# Autodesk Inventor assembly: MechanumChassis
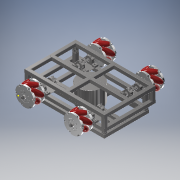
[picture p0: Inventor's stored thumbnail of the model, 180x180]
Saved by Autodesk Inventor 2018 (Build 220112000, 112)
## iProperties
Created: 2017-10-18
Part Number: MechanumChassis
Document SubType Name: Weldment
Designer: Bryce Richards
Mass: 42172.1 g
Surface Area: 44852.8 cm^2
Volume: 5448.29 cm^3
Density: 7.74044 g/cm^3
Weld Material: Steel, Mild, Welded
Author: Bryce Richards
## Documents named in this file (18)
- C:\Users\P136265\Documents\mecanum-cad\MechanumChassis.iam
- C:\Users\P136265\Documents\mecanum-cad\MecanumFrame2.iam
- C:\Users\P136265\Documents\mecanum-cad\PillowAssembly.iam
- C:\Users\P136265\Documents\Inventor\Content Center Files\R2018\en-US\AS 1110\AS 1110 - M8 x 60.ipt
- C:\Users\P136265\Documents\Inventor\Content Center Files\R2018\en-US\AS 1112 (2)\AS 1112 - M8  Type 5.ipt
- C:\Users\P136265\Documents\mecanum-cad\PillowPlate.ipt
- C:\Users\P136265\Documents\mecanum-cad\LiftPlate.iam
- C:\Users\P136265\Documents\mecanum-cad\AlignmentTube.ipt
- C:\Users\P136265\Documents\mecanum-cad\LoadTestBlock.ipt
- C:\Users\P136265\Documents\mecanum-cad\WheelShaft.ipt
- C:\Users\P136265\Documents\mecanum-cad\Mecanum_Assembly.iam
- C:\Users\P136265\Documents\Inventor\Content Center Files\R2018\en-US\ISO 4032(2)\ISO 4032 - M20 - ISO.ipt
- C:\Users\P136265\Documents\mecanum-cad\MechanumChassis\AIP\FEA\cayefugao.fins
- C:\Users\P136265\Documents\mecanum-cad\MechanumChassis\AIP\FEA\cayefugao.fsat
- C:\Users\P136265\Documents\mecanum-cad\MechanumChassis\AIP\FEA\cayefugao.ftes
- C:\Users\P136265\Documents\mecanum-cad\MechanumChassis\AIP\FEA\cayefugao.fwiz
- C:\Users\P136265\Documents\mecanum-cad\MechanumChassis\AIP\FEA\cayefuglc.fmsh
- C:\Users\P136265\Documents\mecanum-cad\MechanumChassis\AIP\FEA\cayefugld.fres
## Components (67 placed, 11 different names)
1. MecanumFrame2:1 [sub-assembly] — Flush:2, Flush:6, Flush:7, Mate:56, Mate:69, Mate:70, Mate:71, Mate:90, Angle:5, Angle:6, Angle:7, Flush:10, Insert:17, Insert:18, Insert:19, Insert:20, Insert:21, Insert:22, Insert:23, Insert:24, Insert:25, Insert:26, Insert:27, Insert:28, Insert:29, Insert:30, Insert:31, Insert:32, Angle:8, Mate:209, Mate:210, Flush:11, Angle:9, Angle:10, Angle:11, Mate:211, Mate:212, Flush:12, Mate:213, Mate:214, Flush:13, Mate:215, Mate:216, Flush:14, Angle:12, Mate:221, Mate:222, Mate:223, Angle:13, Angle:14, Angle:15, Angle:16, Angle:17, Angle:18, Angle:19, Angle:20, Mate:225, Mate:226, Mate:227, Mate:228, Mate:234, Mate:235, Mate:236, Mate:237
2. PillowAssembly:1 [sub-assembly] — Mate:16, Mate:59, Mate:186, Mate:190, Mate:233, Flush:17, Mate:234
3. PillowAssembly:2 [sub-assembly] — Mate:13, Mate:62, Mate:178, Mate:180, Mate:231, Mate:232, Mate:235
4. PillowAssembly:3 [sub-assembly] — Mate:15, Mate:63, Mate:64, Mate:202, Mate:206, Mate:230, Flush:16, Mate:236
5. PillowAssembly:4 [sub-assembly] — Mate:51, Mate:52, Mate:53, Mate:194, Mate:196, Mate:229, Flush:15, Mate:237
6. PillowAssembly:5 [sub-assembly] — Mate:13, Flush:2, Mate:60, Mate:61, Mate:182, Mate:184, Mate:253
7. PillowAssembly:6 [sub-assembly] — Mate:15, Mate:65, Flush:10, Mate:204, Mate:208, Mate:251
8. PillowAssembly:7 [sub-assembly] — Flush:6, Mate:16, Mate:57, Mate:58, Mate:188, Mate:192, Mate:257
9. PillowAssembly:8 [sub-assembly] — Flush:7, Mate:51, Mate:54, Mate:198, Mate:200, Mate:255
10. PillowPlate:1 — Mate:52, Mate:53, Mate:54, Mate:56
11. PillowPlate:2 — Mate:57, Mate:58, Mate:59, Mate:71
12. PillowPlate:3 — Mate:60, Mate:61, Mate:62, Mate:70
13. PillowPlate:4 — Mate:63, Mate:64, Mate:65, Mate:69
14. LiftPlate:1 [sub-assembly] — Angle:13, Angle:14, Angle:15, Angle:16, Angle:17, Angle:18, Angle:19, Angle:20, Mate:225, Mate:226, Mate:227, Mate:228
15. AS 1110 - Metric M8 x 60:17 — Insert:17, Mate:179
16. AS 1110 - Metric M8 x 60:18 — Insert:18, Mate:177
17. AS 1110 - Metric M8 x 60:19 — Insert:19, Mate:183
18. AS 1110 - Metric M8 x 60:20 — Insert:20, Mate:181
19. AS 1110 - Metric M8 x 60:21 — Insert:21, Mate:187
20. AS 1110 - Metric M8 x 60:22 — Insert:22, Mate:191
21. AS 1110 - Metric M8 x 60:23 — Insert:23, Mate:189
22. AS 1110 - Metric M8 x 60:24 — Insert:24, Mate:185
23. AS 1110 - Metric M8 x 60:25 — Insert:25, Mate:199
24. AS 1110 - Metric M8 x 60:26 — Insert:26, Mate:197
25. AS 1110 - Metric M8 x 60:27 — Insert:27, Mate:195
26. AS 1110 - Metric M8 x 60:28 — Insert:28, Mate:193
27. AS 1110 - Metric M8 x 60:29 — Insert:29, Mate:201
28. AS 1110 - Metric M8 x 60:30 — Insert:30, Mate:203
29. AS 1110 - Metric M8 x 60:31 — Insert:31, Mate:207
30. AS 1110 - Metric M8 x 60:32 — Insert:32, Mate:205
31. AS 1112 (2) - Metric M8  Type 5:17 — Mate:177, Mate:178
32. AS 1112 (2) - Metric M8  Type 5:18 — Mate:179, Mate:180
33. AS 1112 (2) - Metric M8  Type 5:19 — Mate:181, Mate:182
34. AS 1112 (2) - Metric M8  Type 5:20 — Mate:183, Mate:184
35. AS 1112 (2) - Metric M8  Type 5:21 — Mate:185, Mate:186
36. AS 1112 (2) - Metric M8  Type 5:22 — Mate:187, Mate:188
37. AS 1112 (2) - Metric M8  Type 5:23 — Mate:189, Mate:190
38. AS 1112 (2) - Metric M8  Type 5:24 — Mate:191, Mate:192
39. AS 1112 (2) - Metric M8  Type 5:25 — Mate:193, Mate:194
40. AS 1112 (2) - Metric M8  Type 5:26 — Mate:195, Mate:196
41. AS 1112 (2) - Metric M8  Type 5:27 — Mate:197, Mate:198
42. AS 1112 (2) - Metric M8  Type 5:28 — Mate:199, Mate:200
43. AS 1112 (2) - Metric M8  Type 5:29 — Mate:201, Mate:202
44. AS 1112 (2) - Metric M8  Type 5:30 — Mate:203, Mate:204
45. AS 1112 (2) - Metric M8  Type 5:31 — Mate:205, Mate:206
46. AS 1112 (2) - Metric M8  Type 5:32 — Mate:207, Mate:208
47. LoadTestBlock:1 — Angle:12, Mate:221, Mate:222, Mate:223
48. AlignmentTube:1 — Angle:10, Mate:213, Mate:214, Flush:13
49. AlignmentTube:2 — Angle:8, Mate:209, Mate:210, Flush:11
50. AlignmentTube:3 — Angle:11, Mate:215, Mate:216, Flush:14
51. AlignmentTube:4 — Angle:9, Mate:211, Mate:212, Flush:12
52. WheelShaft:1 — Mate:233, Flush:17, Angle:23, Angle:26, Mate:240, Flush:20, Mate:244, Mate:256
53. WheelShaft:2 — Mate:231, Mate:232, Angle:22, Angle:27, Mate:241, Flush:21, Mate:242, Mate:252
54. WheelShaft:3 — Mate:230, Flush:16, Angle:21, Angle:22, Angle:23, Angle:25, Mate:239, Flush:19, Mate:246, Mate:250
55. WheelShaft:4 — Mate:229, Flush:15, Angle:21, Angle:24, Mate:238, Flush:18, Mate:248, Mate:254
56. Mecanum_Assembly:1 [sub-assembly] — Angle:27, Mate:241, Flush:21, Mate:243
57. Mecanum_Assembly:2 [sub-assembly] — Angle:26, Mate:240, Flush:20, Mate:245
58. Mecanum_Assembly:3 [sub-assembly] — Angle:25, Mate:239, Flush:19, Mate:247
59. Mecanum_Assembly:4 [sub-assembly] — Angle:24, Mate:238, Flush:18, Mate:249
60. ISO 4032 M20:1 — Mate:242, Mate:243
61. ISO 4032 M20:2 — Mate:244, Mate:245
62. ISO 4032 M20:3 — Mate:246, Mate:247
63. ISO 4032 M20:4 — Mate:248, Mate:249
64. ISO 4032 M20:5 — Mate:250, Mate:251
65. ISO 4032 M20:6 — Mate:252, Mate:253
66. ISO 4032 M20:7 — Mate:254, Mate:255
67. ISO 4032 M20:8 — Mate:256, Mate:257
## Relationships (151: Mate 97, Angle 23, Insert 16, Flush 15)
- Mate:13: PillowAssembly:2 ↔ PillowAssembly:5
- Flush:2: MecanumFrame2:1 ↔ PillowAssembly:5
- Mate:15: PillowAssembly:3 ↔ PillowAssembly:6
- Flush:6: MecanumFrame2:1 ↔ PillowAssembly:7
- Mate:16: PillowAssembly:1 ↔ PillowAssembly:7
- Flush:7: MecanumFrame2:1 ↔ PillowAssembly:8
- Mate:51: PillowAssembly:4 ↔ PillowAssembly:8
- Mate:52: PillowAssembly:4 ↔ PillowPlate:1
- Mate:53: PillowAssembly:4 ↔ PillowPlate:1
- Mate:54: PillowAssembly:8 ↔ PillowPlate:1
- Mate:56: MecanumFrame2:1 ↔ PillowPlate:1
- Mate:57: PillowAssembly:7 ↔ PillowPlate:2
- Mate:58: PillowAssembly:7 ↔ PillowPlate:2
- Mate:59: PillowAssembly:1 ↔ PillowPlate:2
- Mate:60: PillowAssembly:5 ↔ PillowPlate:3
- Mate:61: PillowAssembly:5 ↔ PillowPlate:3
- Mate:62: PillowAssembly:2 ↔ PillowPlate:3
- Mate:63: PillowAssembly:3 ↔ PillowPlate:4
- Mate:64: PillowAssembly:3 ↔ PillowPlate:4
- Mate:65: PillowAssembly:6 ↔ PillowPlate:4
- Mate:69: MecanumFrame2:1 ↔ PillowPlate:4
- Mate:70: MecanumFrame2:1 ↔ PillowPlate:3
- Mate:71: MecanumFrame2:1 ↔ PillowPlate:2
- Mate:90: MecanumFrame2:1
- Angle:5 (0 deg): MecanumFrame2:1
- Angle:6 (0 deg): MecanumFrame2:1
- Angle:7 (0 deg): MecanumFrame2:1
- Flush:10: MecanumFrame2:1 ↔ PillowAssembly:6
- Insert:17: MecanumFrame2:1 ↔ AS 1110 - Metric M8 x 60:17
- Insert:18: MecanumFrame2:1 ↔ AS 1110 - Metric M8 x 60:18
- Insert:19: MecanumFrame2:1 ↔ AS 1110 - Metric M8 x 60:19
- Insert:20: MecanumFrame2:1 ↔ AS 1110 - Metric M8 x 60:20
- Insert:21: MecanumFrame2:1 ↔ AS 1110 - Metric M8 x 60:21
- Insert:22: MecanumFrame2:1 ↔ AS 1110 - Metric M8 x 60:22
- Insert:23: MecanumFrame2:1 ↔ AS 1110 - Metric M8 x 60:23
- Insert:24: MecanumFrame2:1 ↔ AS 1110 - Metric M8 x 60:24
- Insert:25: MecanumFrame2:1 ↔ AS 1110 - Metric M8 x 60:25
- Insert:26: MecanumFrame2:1 ↔ AS 1110 - Metric M8 x 60:26
- Insert:27: MecanumFrame2:1 ↔ AS 1110 - Metric M8 x 60:27
- Insert:28: MecanumFrame2:1 ↔ AS 1110 - Metric M8 x 60:28
- Insert:29: MecanumFrame2:1 ↔ AS 1110 - Metric M8 x 60:29
- Insert:30: MecanumFrame2:1 ↔ AS 1110 - Metric M8 x 60:30
- Insert:31: MecanumFrame2:1 ↔ AS 1110 - Metric M8 x 60:31
- Insert:32: MecanumFrame2:1 ↔ AS 1110 - Metric M8 x 60:32
- Mate:177: AS 1110 - Metric M8 x 60:18 ↔ AS 1112 (2) - Metric M8  Type 5:17
- Mate:178: PillowAssembly:2 ↔ AS 1112 (2) - Metric M8  Type 5:17
- Mate:179: AS 1110 - Metric M8 x 60:17 ↔ AS 1112 (2) - Metric M8  Type 5:18
- Mate:180: PillowAssembly:2 ↔ AS 1112 (2) - Metric M8  Type 5:18
- Mate:181: AS 1110 - Metric M8 x 60:20 ↔ AS 1112 (2) - Metric M8  Type 5:19
- Mate:182: PillowAssembly:5 ↔ AS 1112 (2) - Metric M8  Type 5:19
- Mate:183: AS 1110 - Metric M8 x 60:19 ↔ AS 1112 (2) - Metric M8  Type 5:20
- Mate:184: PillowAssembly:5 ↔ AS 1112 (2) - Metric M8  Type 5:20
- Mate:185: AS 1110 - Metric M8 x 60:24 ↔ AS 1112 (2) - Metric M8  Type 5:21
- Mate:186: PillowAssembly:1 ↔ AS 1112 (2) - Metric M8  Type 5:21
- Mate:187: AS 1110 - Metric M8 x 60:21 ↔ AS 1112 (2) - Metric M8  Type 5:22
- Mate:188: PillowAssembly:7 ↔ AS 1112 (2) - Metric M8  Type 5:22
- Mate:189: AS 1110 - Metric M8 x 60:23 ↔ AS 1112 (2) - Metric M8  Type 5:23
- Mate:190: PillowAssembly:1 ↔ AS 1112 (2) - Metric M8  Type 5:23
- Mate:191: AS 1110 - Metric M8 x 60:22 ↔ AS 1112 (2) - Metric M8  Type 5:24
- Mate:192: PillowAssembly:7 ↔ AS 1112 (2) - Metric M8  Type 5:24
- Mate:193: AS 1110 - Metric M8 x 60:28 ↔ AS 1112 (2) - Metric M8  Type 5:25
- Mate:194: PillowAssembly:4 ↔ AS 1112 (2) - Metric M8  Type 5:25
- Mate:195: AS 1110 - Metric M8 x 60:27 ↔ AS 1112 (2) - Metric M8  Type 5:26
- Mate:196: PillowAssembly:4 ↔ AS 1112 (2) - Metric M8  Type 5:26
- Mate:197: AS 1110 - Metric M8 x 60:26 ↔ AS 1112 (2) - Metric M8  Type 5:27
- Mate:198: PillowAssembly:8 ↔ AS 1112 (2) - Metric M8  Type 5:27
- Mate:199: AS 1110 - Metric M8 x 60:25 ↔ AS 1112 (2) - Metric M8  Type 5:28
- Mate:200: PillowAssembly:8 ↔ AS 1112 (2) - Metric M8  Type 5:28
- Mate:201: AS 1110 - Metric M8 x 60:29 ↔ AS 1112 (2) - Metric M8  Type 5:29
- Mate:202: PillowAssembly:3 ↔ AS 1112 (2) - Metric M8  Type 5:29
- Mate:203: AS 1110 - Metric M8 x 60:30 ↔ AS 1112 (2) - Metric M8  Type 5:30
- Mate:204: PillowAssembly:6 ↔ AS 1112 (2) - Metric M8  Type 5:30
- Mate:205: AS 1110 - Metric M8 x 60:32 ↔ AS 1112 (2) - Metric M8  Type 5:31
- Mate:206: PillowAssembly:3 ↔ AS 1112 (2) - Metric M8  Type 5:31
- Mate:207: AS 1110 - Metric M8 x 60:31 ↔ AS 1112 (2) - Metric M8  Type 5:32
- Mate:208: PillowAssembly:6 ↔ AS 1112 (2) - Metric M8  Type 5:32
- Angle:8 (0 deg): MecanumFrame2:1 ↔ AlignmentTube:2
- Mate:209: MecanumFrame2:1 ↔ AlignmentTube:2
- Mate:210: MecanumFrame2:1 ↔ AlignmentTube:2
- Flush:11: MecanumFrame2:1 ↔ AlignmentTube:2
- Angle:9 (0 deg): MecanumFrame2:1 ↔ AlignmentTube:4
- Angle:10 (0 deg): MecanumFrame2:1 ↔ AlignmentTube:1
- Angle:11 (0 deg): MecanumFrame2:1 ↔ AlignmentTube:3
- Mate:211: MecanumFrame2:1 ↔ AlignmentTube:4
- Mate:212: MecanumFrame2:1 ↔ AlignmentTube:4
- Flush:12: MecanumFrame2:1 ↔ AlignmentTube:4
- Mate:213: MecanumFrame2:1 ↔ AlignmentTube:1
- Mate:214: MecanumFrame2:1 ↔ AlignmentTube:1
- Flush:13: MecanumFrame2:1 ↔ AlignmentTube:1
- Mate:215: MecanumFrame2:1 ↔ AlignmentTube:3
- Mate:216: MecanumFrame2:1 ↔ AlignmentTube:3
- Flush:14: MecanumFrame2:1 ↔ AlignmentTube:3
- Angle:12 (0 deg): MecanumFrame2:1 ↔ LoadTestBlock:1
- Mate:221: MecanumFrame2:1 ↔ LoadTestBlock:1
- Mate:222 (232.5 mm): MecanumFrame2:1 ↔ LoadTestBlock:1
- Mate:223 (382.5 mm): MecanumFrame2:1 ↔ LoadTestBlock:1
- Angle:13 (0 deg): MecanumFrame2:1 ↔ LiftPlate:1
- Angle:14 (0 deg): MecanumFrame2:1 ↔ LiftPlate:1
- Angle:15 (0 deg): MecanumFrame2:1 ↔ LiftPlate:1
- Angle:16 (0 deg): MecanumFrame2:1 ↔ LiftPlate:1
- Angle:17 (0 deg): MecanumFrame2:1 ↔ LiftPlate:1
- Angle:18 (0 deg): MecanumFrame2:1 ↔ LiftPlate:1
- Angle:19 (0 deg): MecanumFrame2:1 ↔ LiftPlate:1
- Angle:20 (0 deg): MecanumFrame2:1 ↔ LiftPlate:1
- Mate:225: MecanumFrame2:1 ↔ LiftPlate:1
- Mate:226: MecanumFrame2:1 ↔ LiftPlate:1
- Mate:227: MecanumFrame2:1 ↔ LiftPlate:1
- Mate:228: MecanumFrame2:1 ↔ LiftPlate:1
- Mate:229: PillowAssembly:4 ↔ WheelShaft:4
- Flush:15 (-160 mm): PillowAssembly:4 ↔ WheelShaft:4
- Mate:230: PillowAssembly:3 ↔ WheelShaft:3
- Flush:16 (-160 mm): PillowAssembly:3 ↔ WheelShaft:3
- Mate:231: PillowAssembly:2 ↔ WheelShaft:2
- Mate:232 (15 mm): PillowAssembly:2 ↔ WheelShaft:2
- Mate:233: PillowAssembly:1 ↔ WheelShaft:1
- Flush:17 (-190 mm): PillowAssembly:1 ↔ WheelShaft:1
- Mate:234: MecanumFrame2:1 ↔ PillowAssembly:1
- Mate:235: MecanumFrame2:1 ↔ PillowAssembly:2
- Mate:236: MecanumFrame2:1 ↔ PillowAssembly:3
- Mate:237: MecanumFrame2:1 ↔ PillowAssembly:4
- Angle:21 (0 deg): WheelShaft:3 ↔ WheelShaft:4
- Angle:22 (0 deg): WheelShaft:2 ↔ WheelShaft:3
- Angle:23 (0 deg): WheelShaft:1 ↔ WheelShaft:3
- Angle:24 (0 deg): WheelShaft:4 ↔ Mecanum_Assembly:4
- Mate:238: WheelShaft:4 ↔ Mecanum_Assembly:4
- Flush:18: WheelShaft:4 ↔ Mecanum_Assembly:4
- Angle:25 (0 deg): WheelShaft:3 ↔ Mecanum_Assembly:3
- Mate:239: WheelShaft:3 ↔ Mecanum_Assembly:3
- Flush:19: WheelShaft:3 ↔ Mecanum_Assembly:3
- Angle:26 (0 deg): WheelShaft:1 ↔ Mecanum_Assembly:2
- Mate:240: WheelShaft:1 ↔ Mecanum_Assembly:2
- Flush:20: WheelShaft:1 ↔ Mecanum_Assembly:2
- Angle:27 (0 deg): WheelShaft:2 ↔ Mecanum_Assembly:1
- Mate:241: WheelShaft:2 ↔ Mecanum_Assembly:1
- Flush:21: WheelShaft:2 ↔ Mecanum_Assembly:1
- Mate:242: WheelShaft:2 ↔ ISO 4032 M20:1
- Mate:243: Mecanum_Assembly:1 ↔ ISO 4032 M20:1
- Mate:244: WheelShaft:1 ↔ ISO 4032 M20:2
- Mate:245: Mecanum_Assembly:2 ↔ ISO 4032 M20:2
- Mate:246: WheelShaft:3 ↔ ISO 4032 M20:3
- Mate:247: Mecanum_Assembly:3 ↔ ISO 4032 M20:3
- Mate:248: WheelShaft:4 ↔ ISO 4032 M20:4
- Mate:249: Mecanum_Assembly:4 ↔ ISO 4032 M20:4
- Mate:250: WheelShaft:3 ↔ ISO 4032 M20:5
- Mate:251: PillowAssembly:6 ↔ ISO 4032 M20:5
- Mate:252: WheelShaft:2 ↔ ISO 4032 M20:6
- Mate:253: PillowAssembly:5 ↔ ISO 4032 M20:6
- Mate:254: WheelShaft:4 ↔ ISO 4032 M20:7
- Mate:255: PillowAssembly:8 ↔ ISO 4032 M20:7
- Mate:256: WheelShaft:1 ↔ ISO 4032 M20:8
- Mate:257: PillowAssembly:7 ↔ ISO 4032 M20:8
## Named parameters: sa_0 = 2.05613e-08, sa_1 = -2.31309e-08, sa_2 = 588000
note: some values were not read from the file. Shown as the stored number, unit unknown: "sa_0", "sa_1", "sa_2".
